# Autodesk Inventor assembly: Montagem_01
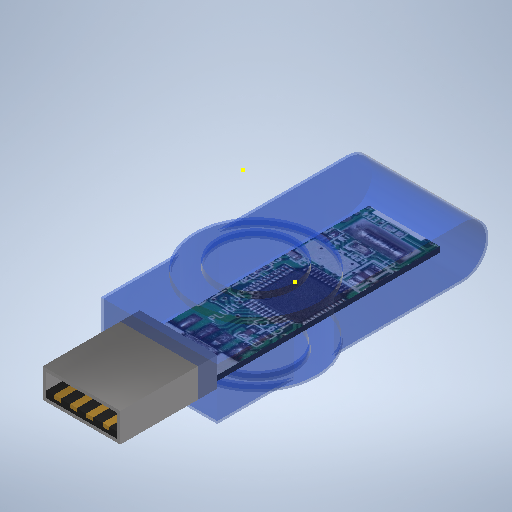
[picture p0: Inventor's stored thumbnail of the model, 512x512]
Saved by Autodesk Inventor 2025 (Build 290162000, 162)
## iProperties
Created: 2024-04-22
Part Number: Montagem_01
Document SubType Name: Assembly
Designer: 082220022
Author: 082220022
## Documents named in this file (5)
- C:\Users\Testwork\Desktop\Projetos Inventor\Montagem_01.iam
- C:\Users\Testwork\Desktop\Projetos Inventor\capa.ipt
- C:\Users\Testwork\Desktop\Projetos Inventor\Pen2.ipt
- C:\Users\Testwork\Desktop\Projetos Inventor\pen3_barra.ipt
- C:\Users\Testwork\Desktop\Projetos Inventor\Pendrive.ipt
## Components (7 placed, 4 different names)
1. capa:1 — Coincidente:4, Alinhado:4, Coincidente:5, Alinhado:5, Coincidente:6, Coincidente:7
2. Pen2:1 — Coincidente:2, Alinhado:3, Coincidente:3, Coincidente:4, Alinhado:4, Coincidente:5
3. Pendrive:1 — Coincidente:1, Alinhado:1, Alinhado:2, Alinhado:5, Coincidente:6, Coincidente:7
4. pen3_barra:1 — Coincidente:2, Alinhado:3, Coincidente:3
5. pen3_barra:2
6. pen3_barra:3
7. pen3_barra:4
## Component patterns: (4 elements, first: pen3_barra:1)
## Relationships (12: Mate 7, Flush 5)
- Coincidente:1 [Mate]: Pendrive:1
- Alinhado:1 [Flush]: Pendrive:1
- Alinhado:2 [Flush]: Pendrive:1
- Coincidente:2 [Mate]: Pen2:1 ↔ pen3_barra:1
- Alinhado:3 [Flush]: Pen2:1 ↔ pen3_barra:1
- Coincidente:3 [Mate]: Pen2:1 ↔ pen3_barra:1
- Coincidente:4 [Mate]: capa:1 ↔ Pen2:1
- Alinhado:4 [Flush]: capa:1 ↔ Pen2:1
- Coincidente:5 [Mate]: capa:1 ↔ Pen2:1
- Alinhado:5 [Flush] (-12 mm): capa:1 ↔ Pendrive:1
- Coincidente:6 [Mate]: capa:1 ↔ Pendrive:1
- Coincidente:7 [Mate]: capa:1 ↔ Pendrive:1
